# Autodesk Inventor assembly: Dog Shifter Reverse
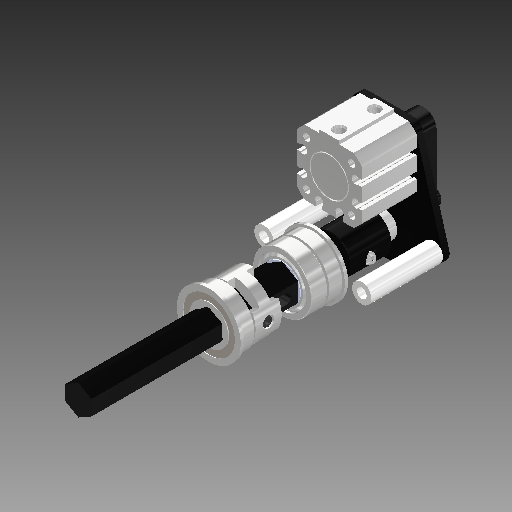
[picture p0: Inventor's stored thumbnail of the model, 512x512]
Saved by Autodesk Inventor 2022 (Build 260153000, 153)
## iProperties
Created: 2021-04-11
Part Number: Dog Shifter Reverse
Document SubType Name: Assembly
Designer: Cal
Author: Cal
## Documents named in this file (10)
- E:\Middleton Robotics\Collaborative Robots\Collaborative Part Library\Power Transfer\Shifters\Dog Shifter Reverse.iam
- E:\Middleton Robotics\Collaborative Robots\Collaborative Part Library\Power Transfer\Shifters\Dog Shifter Stack Reverse.ipt
- E:\Middleton Robotics\Collaborative Robots\Collaborative Part Library\Power Transfer\Shifters\Dog Shifter Coupler Spacer.ipt
- E:\Middleton Robotics\Collaborative Robots\Collaborative Part Library\Hardware\Spacers & Standoffs\Nylon Unthreaded Spacer (No. 10 x 1.375Lg x 0.375OD).ipt
- C:\Users\Cal\Desktop\Robotics\Design\CollabPartsLib\Hardware\Spacers & Standoffs.ipt
- E:\Middleton Robotics\Collaborative Robots\Collaborative Part Library\Pneumatics\.5in .75 Pancake Air Cylinder 217-2778.ipt
- E:\Middleton Robotics\Collaborative Robots\Collaborative Part Library\Power Transfer\Shifters\Dog Shifter Reverse Plate.ipt
- E:\Middleton Robotics\Collaborative Robots\Collaborative Part Library\Power Transfer\Shifters\Dog Shifter Reverse Connector Plate.ipt
- E:\Middleton Robotics\Collaborative Robots\Collaborative Part Library\Hardware\Machine Screws\10-32 UNFx1.375 Socket Head Cap Screw.ipt
- C:\Users\Cal\Desktop\Robotics\Design\CollabPartsLib\Hardware\Machine Screws.ipt
## Components (8 placed, 7 different names)
1. Dog Shifter Stack Reverse:1 — Insert:1, Mate:1, Mate:3, Flush:3
2. Dog Shifter Coupler Spacer:1 — Insert:1
3. Nylon Unthreaded Spacer (No. 10 x 1.375Lg x 0.375OD):1 — Flush:1, Flush:2, Angle:1, Mate:1, Mate:2, Mate:3, Flush:3, Insert:2
4. Nylon Unthreaded Spacer (No. 10 x 1.375Lg x 0.375OD):2 — Flush:1, Flush:2, Mate:2, Mate:4
5. .5in .75 Pancake Air Cylinder 217-2778:1 — Insert:3, Mate:5, Insert:4
6. Dog Shifter Reverse Plate:1 — Insert:2, Mate:4, Insert:3, Mate:5, Mate:6
7. Dog Shifter Reverse Connector Plate:1 — Insert:4, Mate:6, Insert:5
8. Actually maybe 10-24 according to 3846 10-32 UNFx1.375 Socket Head Cap Screw:1 — Insert:5
## Relationships (15: Mate 6, Insert 5, Flush 3, Angle 1)
- Insert:1: Dog Shifter Stack Reverse:1 ↔ Dog Shifter Coupler Spacer:1
- Flush:1: Nylon Unthreaded Spacer (No. 10 x 1.375Lg x 0.375OD):1 ↔ Nylon Unthreaded Spacer (No. 10 x 1.375Lg x 0.375OD):2
- Flush:2: Nylon Unthreaded Spacer (No. 10 x 1.375Lg x 0.375OD):1 ↔ Nylon Unthreaded Spacer (No. 10 x 1.375Lg x 0.375OD):2
- Angle:1 (0 deg): Nylon Unthreaded Spacer (No. 10 x 1.375Lg x 0.375OD):1
- Mate:1: Dog Shifter Stack Reverse:1 ↔ Nylon Unthreaded Spacer (No. 10 x 1.375Lg x 0.375OD):1
- Mate:2 (47.625 mm): Nylon Unthreaded Spacer (No. 10 x 1.375Lg x 0.375OD):1 ↔ Nylon Unthreaded Spacer (No. 10 x 1.375Lg x 0.375OD):2
- Mate:3 (23.8125 mm): Dog Shifter Stack Reverse:1 ↔ Nylon Unthreaded Spacer (No. 10 x 1.375Lg x 0.375OD):1
- Flush:3: Dog Shifter Stack Reverse:1 ↔ Nylon Unthreaded Spacer (No. 10 x 1.375Lg x 0.375OD):1
- Insert:2: Nylon Unthreaded Spacer (No. 10 x 1.375Lg x 0.375OD):1 ↔ Dog Shifter Reverse Plate:1
- Mate:4: Nylon Unthreaded Spacer (No. 10 x 1.375Lg x 0.375OD):2 ↔ Dog Shifter Reverse Plate:1
- Insert:3: .5in .75 Pancake Air Cylinder 217-2778:1 ↔ Dog Shifter Reverse Plate:1
- Mate:5: .5in .75 Pancake Air Cylinder 217-2778:1 ↔ Dog Shifter Reverse Plate:1
- Insert:4: .5in .75 Pancake Air Cylinder 217-2778:1 ↔ Dog Shifter Reverse Connector Plate:1
- Mate:6: Dog Shifter Reverse Plate:1 ↔ Dog Shifter Reverse Connector Plate:1
- Insert:5: Dog Shifter Reverse Connector Plate:1 ↔ Actually maybe 10-24 according to 3846 10-32 UNFx1.375 Socket Head Cap Screw:1
